# Autodesk Inventor assembly: Shoulder_r1
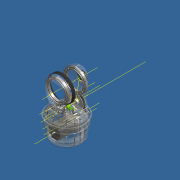
[picture p0: Inventor's stored thumbnail of the model, 180x180]
Saved by Autodesk Inventor 2016 (Build 200138000, 138)
## iProperties
Created: 2015-01-06
Part Number: Shoulder_r1
Document SubType Name: Assembly
Designer: 4ndreas
Mass: 7957.81 g
Surface Area: 6736.07 cm^2
Volume: 2402.06 cm^3
Density: 3.31292 g/cm^3
Parent: R1
Author: 4ndreas
## Documents named in this file (35)
- C:\Users\4ndreas\Documents\github\Mantis-Robot-Arm\MantisRobotArm\Workspace\_assemblys\Shoulder_r1.iam
- C:\Users\4ndreas\Documents\github\Mantis-Robot-Arm\MantisRobotArm\Workspace\_assemblys\Shoulder\Konstruktions-Assistent\Übertragung des Zahnriemens1.iam
- C:\Users\4ndreas\Documents\github\Mantis-Robot-Arm\MantisRobotArm\Libraries\Content Center Files\de-DE\DIN 125-1  A\DIN 125 - A 4,3.ipt
- C:\Users\4ndreas\Documents\github\Mantis-Robot-Arm\MantisRobotArm\Libraries\Content Center Files\de-DE\DIN BEARING(1)\DIN 625 SKF - SKF 624.ipt
- C:\Users\4ndreas\Documents\github\Mantis-Robot-Arm\MantisRobotArm\Libraries\Content Center Files\de-DE\DIN 934\DIN 934 - M4 x 0,7.ipt
- C:\Users\4ndreas\Documents\github\Mantis-Robot-Arm\MantisRobotArm\Workspace\_assemblys\Shoulder\Konstruktions-Assisten2\Übertragung des Zahnriemens1.iam
- C:\Users\4ndreas\Documents\github\Mantis-Robot-Arm\MantisRobotArm\Libraries\Content Center Files\de-DE\DIN BEARING(1)\DIN 625 SKF - SKF 61818.ipt
- C:\Users\4ndreas\Documents\github\Mantis-Robot-Arm\MantisRobotArm\Workspace\_misc parts\Shoulder_basis_N24.ipt
- C:\Users\4ndreas\Documents\github\Mantis-Robot-Arm\MantisRobotArm\Workspace\_assemblys\Shoulder\Konstruktions-Assistent\Welle1.iam
- C:\Users\4ndreas\Documents\github\Mantis-Robot-Arm\MantisRobotArm\Libraries\Content Center Files\de-DE\DIN BEARING(1)\DIN 625 SKF - SKF 608.ipt
- C:\Users\4ndreas\Documents\github\Mantis-Robot-Arm\MantisRobotArm\Libraries\Content Center Files\de-DE\DIN 125-1  A\DIN 125 - A 8,4.ipt
- C:\Users\4ndreas\Documents\github\Mantis-Robot-Arm\MantisRobotArm\Workspace\_printed parts\LagerKlemme.ipt
- C:\Users\4ndreas\Documents\github\Mantis-Robot-Arm\MantisRobotArm\Workspace\_metal parts\16221600.ipt
- C:\Users\4ndreas\Documents\github\Mantis-Robot-Arm\MantisRobotArm\Workspace\_metal parts\Synchrone RiemenscheibeT5_z48.ipt
- C:\Users\4ndreas\Documents\github\Mantis-Robot-Arm\MantisRobotArm\Workspace\_metal parts\Alu_Belt_tens.ipt
- C:\Users\4ndreas\Documents\github\Mantis-Robot-Arm\MantisRobotArm\Libraries\Content Center Files\de-DE\DIN 9021\DIN 9021 - 4,3.ipt
- C:\Users\4ndreas\Documents\github\Mantis-Robot-Arm\MantisRobotArm\Workspace\_standard Parts\DIN 912 - M4 x 0,7 x50.ipt
- C:\Users\4ndreas\Documents\github\Mantis-Robot-Arm\MantisRobotArm\Libraries\Content Center Files\de-DE\DIN 912\DIN 912 - M4 x 0,7 x 20 x 18,25.ipt
- C:\Users\4ndreas\Documents\github\Mantis-Robot-Arm\MantisRobotArm\Libraries\Content Center Files\de-DE\DIN 562\DIN 562 - M4 x 7.ipt
- C:\Users\4ndreas\Documents\github\Mantis-Robot-Arm\MantisRobotArm\Libraries\Content Center Files\de-DE\DIN 912\DIN 912 - M4 x 0,7 x 30 x 20.ipt
- C:\Users\4ndreas\Documents\github\Mantis-Robot-Arm\MantisRobotArm\Workspace\_standard Parts\DIN 912 - M4 x 0,7 x 60.ipt
- C:\Users\4ndreas\Documents\github\Mantis-Robot-Arm\MantisRobotArm\Libraries\Content Center Files\de-DE\DIN 7991(2)\DIN 7991 - M3x25.ipt
- C:\Users\4ndreas\Documents\github\Mantis-Robot-Arm\MantisRobotArm\Libraries\Content Center Files\de-DE\DIN 934\DIN 934 - M3 x 0,5.ipt
- C:\Users\4ndreas\Documents\github\Mantis-Robot-Arm\MantisRobotArm\Libraries\Content Center Files\de-DE\DIN 912\DIN 912 - M4 x 0,7 x 40 x 20.ipt
- C:\Users\4ndreas\Documents\github\Mantis-Robot-Arm\MantisRobotArm\Workspace\_standard Parts\Distanzhuelse_M4x20mm.ipt
- C:\Users\4ndreas\Documents\github\Mantis-Robot-Arm\MantisRobotArm\Libraries\Content Center Files\de-DE\DIN 913\DIN 913 - M4 x 4.ipt
- C:\Users\4ndreas\Documents\github\Mantis-Robot-Arm\MantisRobotArm\Libraries\Content Center Files\de-DE\BS EN ISO 13337\ISO 13337 - 3 x 20BS EN ISO.ipt
- C:\Users\4ndreas\Documents\github\Mantis-Robot-Arm\MantisRobotArm\Libraries\Content Center Files\de-DE\BS EN ISO 13337\ISO 13337 - 3 x 26BS EN ISO.ipt
- C:\Users\4ndreas\Documents\github\Mantis-Robot-Arm\MantisRobotArm\Libraries\Content Center Files\de-DE\DIN 711\DIN 711 - 511 20 - 100 x 135 x 25.ipt
- C:\Users\4ndreas\Documents\github\Mantis-Robot-Arm\MantisRobotArm\Workspace\_printed parts\CoverBase_r1.ipt
- C:\Users\4ndreas\Documents\github\Mantis-Robot-Arm\MantisRobotArm\Workspace\_standard Parts\bearing 6830 150x190x20 .ipt
- C:\Users\4ndreas\Documents\github\Mantis-Robot-Arm\MantisRobotArm\Workspace\_motors\Nema24_100.ipt
- C:\Users\4ndreas\Documents\github\Mantis-Robot-Arm\MantisRobotArm\Workspace\_encoder\encoderR1_mini.ipt
- C:\Users\4ndreas\Documents\github\Mantis-Robot-Arm\MantisRobotArm\Workspace\_encoder\encoder_neu.iam
- C:\Users\4ndreas\Documents\github\Mantis-Robot-Arm\MantisRobotArm\Workspace\_metal parts\Nema23_24Mount.ipt
## Components (139 placed, 32 different names)
1. Übertragung des Zahnriemens:1 [sub-assembly] — Passend:1, Passend:12, Passend:49, Passend:138, Fluchtend:18, Passend:147, Passend:173, Passend:195, Passend:228, Passend:229, Passend:410, Passend:411, Passend:422
2. DIN 912 - ersetzt durch DIN EN ISO 4762 M4 x 50:1 — Passend:69, Passend:82, Passend:99, Passend:179, Passend:198, Passend:203, Passend:209, Passend:210
3. DIN 625 SKF SKF 624:1 — Passend:178, Passend:192
4. DIN 625 SKF SKF 624:2 — Passend:177, Passend:186, Passend:188
5. DIN 625 SKF SKF 624:3 — Passend:80, Passend:82, Passend:181
6. DIN 625 SKF SKF 624:4 — Passend:80, Passend:180, Passend:212
7. DIN 125-1 A A 4,3:3 — Passend:193, Passend:219
8. DIN 125-1 A A 4,3:4 — Passend:183
9. DIN 125-1 A A 4,3:6 — Passend:189, Passend:194
10. DIN 934 - ersetzt durch DIN EN 24032/28673/28674 M4:1 — Passend:99, Passend:183
11. Übertragung des Zahnriemens:2 [sub-assembly] — Passend:130, Passend:182
12. Nema24_100:1 — Passend:130, Winkel:10, Passend:174, Passend:175, Passend:255, Passend:459, Passend:460, Passend:464, Passend:465, Passend:466, Passend:467, Passend:469, Passend:471
13. DIN 625 SKF SKF 61818:1 — Passend:138, Passend:142
14. DIN 625 SKF SKF 61818:2 — Passend:144, Fluchtend:17
15. Shoulder_basis_N24:1 — Passend:139, Fluchtend:14, Passend:140, Fluchtend:16, Passend:142, Passend:143, Passend:144, Fluchtend:17, Passend:164, Passend:169, Fluchtend:19, Passend:182, Passend:69, Passend:191, Fluchtend:20, Passend:204, Passend:205, Passend:206, Passend:208, Passend:213, Passend:221, Passend:224, Passend:225, Passend:226, Passend:227, Passend:230, Passend:300, Passend:301, Passend:302, Passend:303, Passend:304, Passend:305, Passend:306, Passend:307, Passend:308, Passend:309, Passend:310, Passend:311, Passend:328, Passend:329, Passend:330, Passend:331, Passend:332, Passend:333, Passend:334, Passend:335, Passend:336, Passend:337, Passend:338, Passend:339, Passend:340, Passend:341, Passend:342, Passend:344, Passend:345, Passend:346, Passend:353, Passend:354, Passend:355, Passend:356, Passend:357, Passend:358, Passend:359, Passend:367, Passend:369, Passend:370, Passend:371, Passend:374, Passend:375, Fluchtend:52, Fluchtend:53, Passend:423, Passend:424, Passend:425, Passend:426, Passend:448, Passend:449, Passend:450, Passend:451, Passend:456
16. CoverBase_r1:1 — Passend:143, Passend:164, Passend:230, Passend:239, Passend:240, Passend:241, Passend:242, Passend:247, Passend:248, Passend:249, Passend:250, Passend:255, Passend:257, Passend:258, Passend:261, Passend:262, Passend:263, Passend:264, Passend:377, Passend:384, Passend:391, Passend:393, Passend:413, Passend:414, Passend:415, Passend:416, Passend:418, Passend:419, Passend:420, Passend:421, Passend:427, Passend:430, Passend:457, Passend:458, Passend:463, Passend:472
17. Welle:1 [sub-assembly] — Fluchtend:18, Passend:147, Passend:153, Passend:154, Passend:155, Passend:165, Passend:166
18. DIN 625 SKF SKF 608:1 — Passend:153, Passend:167, Passend:169
19. DIN 625 SKF SKF 608:3 — Passend:154, Passend:170, Passend:171
20. DIN 625 SKF SKF 608:4 — Passend:155
21. Synchrone RiemenscheibeT5_z48:1 — Passend:165, Passend:172, Passend:407, Passend:408
22. DIN 125-1 A A 8,4:1 — Passend:166, Passend:167, Passend:172
23. DIN 125-1 A A 8,4:2 — Passend:170, Passend:171, Passend:173
24. LagerKlemme:1 — Fluchtend:19, Passend:226, Passend:227, Passend:324, Passend:325, Passend:326, Passend:327
25. 16221600:1 — Passend:174, Passend:175, Passend:409
26. DIN 625 SKF SKF 624:5 — Passend:177, Passend:178, Passend:190
27. DIN 625 SKF SKF 624:6 — Passend:179, Passend:180, Passend:181
28. Alu_Belt_tens:1 — Passend:186, Passend:191, Passend:196, Passend:197, Fluchtend:20, Passend:222
29. DIN 912 - ersetzt durch DIN EN ISO 4762 M4 x 20:1 — Passend:197, Passend:200, Passend:201
30. DIN 912 - ersetzt durch DIN EN ISO 4762 M4 x 20:2 — Passend:196, Passend:199, Passend:202
31. DIN 912 - ersetzt durch DIN EN ISO 4762 M4 x 40:9 — Passend:188, Passend:189, Passend:190, Passend:192, Passend:193, Passend:194, Passend:195, Passend:207, Passend:218
32. DIN 9021 4,3:1 — Passend:198, Passend:203, Passend:204
33. DIN 9021 4,3:2 — Passend:200, Passend:201, Passend:205
34. DIN 9021 4,3:3 — Passend:199, Passend:202, Passend:206
35. DIN 9021 4,3:4 — Passend:207, Passend:208, Passend:220
36. DIN 9021 4,3:5 — Passend:209, Passend:211, Passend:213
37. DIN 934 - ersetzt durch DIN EN 24032/28673/28674 M4:2 — Passend:210, Passend:211, Passend:212
38. DIN 125-1 A A 4,3:7 — Passend:215, Passend:217, Passend:220
39. DIN 125-1 A A 4,3:8 — Passend:214, Passend:215, Passend:216
40. DIN 125-1 A A 4,3:9 — Passend:214, Passend:216, Passend:217, Passend:218, Passend:219
41. DIN 912 - ersetzt durch DIN EN ISO 4762 M4 x 20:3 — Passend:221, Passend:222, Passend:223
42. DIN 934 - ersetzt durch DIN EN 24032/28673/28674 M4:3 — Passend:223, Passend:224, Passend:225
43. DIN 912 - ersetzt durch DIN EN ISO 4762 M4 x 20:4 — Passend:235, Passend:245, Passend:470, Passend:471
44. DIN 912 - ersetzt durch DIN EN ISO 4762 M4 x 20:5 — Passend:237, Passend:243, Passend:468, Passend:469
45. DIN 912 - ersetzt durch DIN EN ISO 4762 M4 x 20:6 — Passend:236, Passend:244
46. DIN 912 - ersetzt durch DIN EN ISO 4762 M4 x 20:7 — Passend:238, Passend:246
47. DIN 125-1 A A 4,3:10 — Passend:238, Passend:239, Passend:246
48. DIN 125-1 A A 4,3:11 — Passend:237, Passend:241, Passend:243
49. DIN 125-1 A A 4,3:12 — Passend:235, Passend:242, Passend:245
50. DIN 125-1 A A 4,3:13 — Passend:236, Passend:240, Passend:244
51. DIN 625 SKF SKF 624:7 — Passend:248, Passend:251, Passend:252
52. DIN 625 SKF SKF 624:8 — Passend:247, Passend:251, Passend:253, Passend:254
53. DIN 125-1 A A 4,3:14 — Passend:249, Passend:250, Passend:252
54. DIN 125-1 A A 4,3:15 — Passend:253, Passend:254
55. DIN 912 - ersetzt durch DIN EN ISO 4762 M4 x 50:9 — Passend:263, Passend:314, Fluchtend:51
56. DIN 912 - ersetzt durch DIN EN ISO 4762 M4 x 40:1 — Passend:262, Passend:313, Passend:384
57. DIN 912 - ersetzt durch DIN EN ISO 4762 M4 x 50:10 — Passend:261, Fluchtend:28, Passend:312
58. DIN 912 - ersetzt durch DIN EN ISO 4762 M4 x 30:5 — Passend:258, Passend:316, Passend:472
59. DIN 912 - ersetzt durch DIN EN ISO 4762 M4 x 50:13 — Passend:257, Fluchtend:28, Passend:317, Passend:377, Fluchtend:59
60. DIN 912 - ersetzt durch DIN EN ISO 4762 M4 x 50:17 — Passend:264, Passend:315, Fluchtend:51, Fluchtend:59
61. DIN 562 M4:1 — Passend:300, Passend:301, Passend:317
62. DIN 562 M4:2 — Passend:302, Passend:303, Passend:316
63. DIN 562 M4:3 — Passend:304, Passend:305, Passend:315
64. DIN 562 M4:4 — Passend:307, Passend:310, Passend:313
65. DIN 562 M4:5 — Passend:306, Passend:311, Passend:312
66. DIN 562 M4:6 — Passend:308, Passend:309, Passend:314
67. DIN 912 - ersetzt durch DIN EN ISO 4762 M4 x 30:1 — Passend:318, Passend:321, Passend:322, Passend:324
68. DIN 912 - ersetzt durch DIN EN ISO 4762 M4 x 30:2 — Passend:319, Passend:320, Passend:323, Passend:326
69. DIN 934 - ersetzt durch DIN EN 24032/28673/28674 M4:12 — Passend:319, Fluchtend:43, Passend:329
70. DIN 934 - ersetzt durch DIN EN 24032/28673/28674 M4:13 — Passend:318, Fluchtend:43, Passend:328, Passend:330
71. DIN 125-1 A A 4,3:16 — Passend:321, Passend:322, Passend:325
72. DIN 125-1 A A 4,3:17 — Passend:320, Passend:323, Passend:327
73. Distanzhuelse_M4x20mm:9 — Passend:333, Passend:339, Passend:342, Passend:347
74. Distanzhuelse_M4x20mm:10 — Passend:334, Passend:340, Passend:341, Passend:351
75. Distanzhuelse_M4x20mm:11 — Passend:331, Passend:335, Passend:338, Passend:349
76. Distanzhuelse_M4x20mm:12 — Passend:332, Passend:336, Passend:337
77. DIN 912 - ersetzt durch DIN EN ISO 4762 M4 x 50:2 — Passend:344, Passend:346
78. DIN 912 - ersetzt durch DIN EN ISO 4762 M4 x 50:3 — Passend:347, Passend:348, Passend:359
79. DIN 912 - ersetzt durch DIN EN ISO 4762 M4 x 50:4 — Passend:348, Passend:353
80. DIN 912 - ersetzt durch DIN EN ISO 4762 M4 x 50:5 — Passend:345, Passend:356
81. DIN 912 - ersetzt durch DIN EN ISO 4762 M4 x 60:16 — Passend:350, Passend:355
82. DIN 912 - ersetzt durch DIN EN ISO 4762 M4 x 60:17 — Passend:349, Passend:350, Passend:357
83. DIN 912 - ersetzt durch DIN EN ISO 4762 M4 x 60:18 — Passend:352, Passend:354
84. DIN 912 - ersetzt durch DIN EN ISO 4762 M4 x 60:19 — Passend:351, Passend:352, Passend:358
85. DIN 912 - ersetzt durch DIN EN ISO 4762 M4 x 40:8 — Passend:386, Passend:388, Passend:389, Passend:390, Passend:391
86. DIN 125-1 A A 4,3:18 — Passend:386, Passend:390, Passend:463
87. DIN 9021 4,3:6 — Passend:387, Passend:388, Passend:393
88. DIN 934 - ersetzt durch DIN EN 24032/28673/28674 M4:14 — Passend:387, Passend:389
89. DIN 913 M4 x 4:1 — Passend:409
90. DIN 913 M4 x 4:2 — Passend:408
91. BS EN ISO 13337 3 x 20:1 — Passend:410
92. BS EN ISO 13337 3 x 26:1 — Passend:407
93. DIN 913 M4 x 4:3 — Passend:411
94. DIN 711 511 20 - 100 x 135 x 25:1 — Passend:413, Passend:414
95. DIN 625 SKF SKF 61818:3 — Passend:415, Passend:416
96. encoderR1_mini:1 — Passend:418, Passend:420, Passend:421
97. encoder_neu:1 [sub-assembly] — Passend:422, Passend:423, Passend:424
98. DIN 912 - ersetzt durch DIN EN ISO 4762 M4 x 60:1 — Passend:425, Passend:426, Fluchtend:62, Fluchtend:66
99. DIN 912 - ersetzt durch DIN EN ISO 4762 M4 x 40:2 — Passend:427, Passend:431
100. DIN 9021 4,3:11 — Passend:430, Fluchtend:61, Fluchtend:73, Fluchtend:74, Fluchtend:75
101. Distanzhuelse_M4x20mm:13 — Passend:431, Fluchtend:60, Fluchtend:67, Fluchtend:68
102. DIN 912 - ersetzt durch DIN EN ISO 4762 M4 x 60:20 — Passend:435, Fluchtend:62, Passend:448
103. DIN 912 - ersetzt durch DIN EN ISO 4762 M4 x 40:3
104. DIN 9021 4,3:12 — Fluchtend:61, Fluchtend:74
105. Distanzhuelse_M4x20mm:14 — Passend:435, Fluchtend:60
106. DIN 912 - ersetzt durch DIN EN ISO 4762 M4 x 60:21 — Passend:451, Fluchtend:64, Fluchtend:65
107. DIN 912 - ersetzt durch DIN EN ISO 4762 M4 x 40:4
108. DIN 9021 4,3:13 — Fluchtend:71
109. Distanzhuelse_M4x20mm:15 — Fluchtend:70
110. DIN 912 - ersetzt durch DIN EN ISO 4762 M4 x 60:22 — Passend:450, Fluchtend:63
111. DIN 912 - ersetzt durch DIN EN ISO 4762 M4 x 40:5
112. DIN 9021 4,3:14 — Fluchtend:72, Fluchtend:73
113. Distanzhuelse_M4x20mm:16 — Fluchtend:69
114. DIN 912 - ersetzt durch DIN EN ISO 4762 M4 x 60:23 — Passend:449, Fluchtend:65, Fluchtend:66
115. DIN 912 - ersetzt durch DIN EN ISO 4762 M4 x 40:6
116. DIN 9021 4,3:15 — Fluchtend:75
117. Distanzhuelse_M4x20mm:17 — Fluchtend:67
118. DIN 912 - ersetzt durch DIN EN ISO 4762 M4 x 60:24 — Passend:456, Fluchtend:63, Fluchtend:64
119. DIN 912 - ersetzt durch DIN EN ISO 4762 M4 x 40:7
120. DIN 9021 4,3:16 — Fluchtend:71, Fluchtend:72
121. Distanzhuelse_M4x20mm:18 — Fluchtend:68, Fluchtend:69, Fluchtend:70
122. DIN 912 - ersetzt durch DIN EN ISO 4762 M4 x 30:3 — Passend:458, Passend:460, Passend:461
123. DIN 912 - ersetzt durch DIN EN ISO 4762 M4 x 30:4 — Passend:457, Passend:459, Passend:462
124. DIN 934 - ersetzt durch DIN EN 24032/28673/28674 M4:19 — Passend:461, Fluchtend:76, Fluchtend:77
125. DIN 934 - ersetzt durch DIN EN 24032/28673/28674 M4:20 — Passend:462, Fluchtend:76, Fluchtend:77
126. Nema23_24Mount:1 — Passend:464, Passend:465, Passend:466
127. Nema23_24Mount:2 — Passend:467, Passend:468, Passend:470
128. DIN 934 - ersetzt durch DIN EN 24032/28673/28674 M3:1 — Passend:368, Passend:369, Passend:370
129. DIN 7991 M3x25:1 — Passend:367, Fluchtend:52, Passend:368
130. DIN 934 - ersetzt durch DIN EN 24032/28673/28674 M3:2
131. DIN 7991 M3x25:2
132. DIN 934 - ersetzt durch DIN EN 24032/28673/28674 M3:3
133. DIN 7991 M3x25:3
134. DIN 7991 M3x25:8 — Passend:371, Passend:373, Fluchtend:53
135. DIN 934 - ersetzt durch DIN EN 24032/28673/28674 M3:8 — Passend:373, Passend:374, Passend:375
136. DIN 7991 M3x25:9
137. DIN 934 - ersetzt durch DIN EN 24032/28673/28674 M3:9
138. DIN 7991 M3x25:10
139. DIN 934 - ersetzt durch DIN EN 24032/28673/28674 M3:10
## Component patterns: (3 elements, first: DIN 934 - ersetzt durch DIN EN 24032/28673/28674 M3:1 + DIN 7991 M3x25:1), (3 elements, first: DIN 7991 M3x25:8 + DIN 934 - ersetzt durch DIN EN 24032/28673/28674 M3:8)
## Relationships (287: Mate 254, Flush 32, Angle 1)
- Passend:1 [Mate]: Übertragung des Zahnriemens:1
- Passend:4 [Mate]
- Passend:12 [Mate]: Übertragung des Zahnriemens:1
- Passend:49 [Mate]: Übertragung des Zahnriemens:1
- Passend:62 [Mate]
- Passend:63 [Mate]
- Passend:69 [Mate]: DIN 912 - ersetzt durch DIN EN ISO 4762 M4 x 50:1 ↔ Shoulder_basis_N24:1
- Passend:80 [Mate]: DIN 625 SKF SKF 624:3 ↔ DIN 625 SKF SKF 624:4
- Passend:82 [Mate]: DIN 912 - ersetzt durch DIN EN ISO 4762 M4 x 50:1 ↔ DIN 625 SKF SKF 624:3
- [Mate]: DIN 912 - ersetzt durch DIN EN ISO 4762 M4 x 50:1 ↔ DIN 125-1 A A 4,3:4
- [Mate]: DIN 625 SKF SKF 624:3 ↔ DIN 125-1 A A 4,3:4
- [Mate]: DIN 625 SKF SKF 624:2 ↔ DIN 125-1 A A 4,3:6
- [Mate]: DIN 625 SKF SKF 624:1 ↔ DIN 125-1 A A 4,3:3
- Passend:99 [Mate]: DIN 912 - ersetzt durch DIN EN ISO 4762 M4 x 50:1 ↔ DIN 934 - ersetzt durch DIN EN 24032/28673/28674 M4:1
- Fluchtend:12 [Flush] (43 mm)
- Fluchtend:13 [Flush] (20 mm)
- Passend:130 [Mate]: Übertragung des Zahnriemens:2 ↔ Nema24_100:1
- Winkel:10 [Angle] (0 deg): Nema24_100:1
- Passend:138 [Mate]: Übertragung des Zahnriemens:1 ↔ DIN 625 SKF SKF 61818:1
- Passend:139 [Mate]: Shoulder_basis_N24:1
- Fluchtend:14 [Flush]: Shoulder_basis_N24:1
- Passend:140 [Mate]: Shoulder_basis_N24:1
- Fluchtend:16 [Flush]: Shoulder_basis_N24:1
- Passend:142 [Mate]: DIN 625 SKF SKF 61818:1 ↔ Shoulder_basis_N24:1
- Passend:143 [Mate]: Shoulder_basis_N24:1 ↔ CoverBase_r1:1
- Passend:144 [Mate]: DIN 625 SKF SKF 61818:2 ↔ Shoulder_basis_N24:1
- Fluchtend:17 [Flush]: DIN 625 SKF SKF 61818:2 ↔ Shoulder_basis_N24:1
- Fluchtend:18 [Flush] (-10 mm): Übertragung des Zahnriemens:1 ↔ Welle:1
- Passend:147 [Mate]: Übertragung des Zahnriemens:1 ↔ Welle:1
- Passend:153 [Mate]: Welle:1 ↔ DIN 625 SKF SKF 608:1
- Passend:154 [Mate]: Welle:1 ↔ DIN 625 SKF SKF 608:3
- Passend:155 [Mate]: Welle:1 ↔ DIN 625 SKF SKF 608:4
- Passend:164 [Mate]: Shoulder_basis_N24:1 ↔ CoverBase_r1:1
- Passend:165 [Mate]: Welle:1 ↔ Synchrone RiemenscheibeT5_z48:1
- Passend:166 [Mate]: Welle:1 ↔ DIN 125-1 A A 8,4:1
- Passend:167 [Mate]: DIN 625 SKF SKF 608:1 ↔ DIN 125-1 A A 8,4:1
- Passend:169 [Mate]: Shoulder_basis_N24:1 ↔ DIN 625 SKF SKF 608:1
- Passend:170 [Mate]: DIN 625 SKF SKF 608:3 ↔ DIN 125-1 A A 8,4:2
- Passend:171 [Mate]: DIN 625 SKF SKF 608:3 ↔ DIN 125-1 A A 8,4:2
- Passend:172 [Mate]: Synchrone RiemenscheibeT5_z48:1 ↔ DIN 125-1 A A 8,4:1
- Passend:173 [Mate] (0.5 mm): Übertragung des Zahnriemens:1 ↔ DIN 125-1 A A 8,4:2
- Fluchtend:19 [Flush]: Shoulder_basis_N24:1 ↔ LagerKlemme:1
- Passend:174 [Mate]: Nema24_100:1 ↔ 16221600:1
- Passend:175 [Mate] (0.5 mm): Nema24_100:1 ↔ 16221600:1
- Passend:177 [Mate]: DIN 625 SKF SKF 624:2 ↔ DIN 625 SKF SKF 624:5
- Passend:178 [Mate]: DIN 625 SKF SKF 624:1 ↔ DIN 625 SKF SKF 624:5
- Passend:179 [Mate]: DIN 912 - ersetzt durch DIN EN ISO 4762 M4 x 50:1 ↔ DIN 625 SKF SKF 624:6
- Passend:180 [Mate]: DIN 625 SKF SKF 624:4 ↔ DIN 625 SKF SKF 624:6
- Passend:181 [Mate]: DIN 625 SKF SKF 624:3 ↔ DIN 625 SKF SKF 624:6
- Passend:182 [Mate]: Übertragung des Zahnriemens:2 ↔ Shoulder_basis_N24:1
- Passend:183 [Mate]: DIN 125-1 A A 4,3:4 ↔ DIN 934 - ersetzt durch DIN EN 24032/28673/28674 M4:1
- Passend:186 [Mate]: DIN 625 SKF SKF 624:2 ↔ Alu_Belt_tens:1
- Passend:188 [Mate]: DIN 625 SKF SKF 624:2 ↔ DIN 912 - ersetzt durch DIN EN ISO 4762 M4 x 40:9
- Passend:189 [Mate]: DIN 125-1 A A 4,3:6 ↔ DIN 912 - ersetzt durch DIN EN ISO 4762 M4 x 40:9
- Passend:190 [Mate]: DIN 625 SKF SKF 624:5 ↔ DIN 912 - ersetzt durch DIN EN ISO 4762 M4 x 40:9
- Passend:191 [Mate]: Shoulder_basis_N24:1 ↔ Alu_Belt_tens:1
- Passend:192 [Mate]: DIN 625 SKF SKF 624:1 ↔ DIN 912 - ersetzt durch DIN EN ISO 4762 M4 x 40:9
- Passend:193 [Mate]: DIN 125-1 A A 4,3:3 ↔ DIN 912 - ersetzt durch DIN EN ISO 4762 M4 x 40:9
- Passend:194 [Mate]: DIN 125-1 A A 4,3:6 ↔ DIN 912 - ersetzt durch DIN EN ISO 4762 M4 x 40:9
- Passend:195 [Mate]: Übertragung des Zahnriemens:1 ↔ DIN 912 - ersetzt durch DIN EN ISO 4762 M4 x 40:9
- Passend:196 [Mate]: Alu_Belt_tens:1 ↔ DIN 912 - ersetzt durch DIN EN ISO 4762 M4 x 20:2
- Passend:197 [Mate]: Alu_Belt_tens:1 ↔ DIN 912 - ersetzt durch DIN EN ISO 4762 M4 x 20:1
- Fluchtend:20 [Flush]: Shoulder_basis_N24:1 ↔ Alu_Belt_tens:1
- Passend:198 [Mate]: DIN 912 - ersetzt durch DIN EN ISO 4762 M4 x 50:1 ↔ DIN 9021 4,3:1
- Passend:199 [Mate]: DIN 912 - ersetzt durch DIN EN ISO 4762 M4 x 20:2 ↔ DIN 9021 4,3:3
- Passend:200 [Mate]: DIN 912 - ersetzt durch DIN EN ISO 4762 M4 x 20:1 ↔ DIN 9021 4,3:2
- Passend:201 [Mate]: DIN 912 - ersetzt durch DIN EN ISO 4762 M4 x 20:1 ↔ DIN 9021 4,3:2
- Passend:202 [Mate]: DIN 912 - ersetzt durch DIN EN ISO 4762 M4 x 20:2 ↔ DIN 9021 4,3:3
- Passend:203 [Mate]: DIN 912 - ersetzt durch DIN EN ISO 4762 M4 x 50:1 ↔ DIN 9021 4,3:1
- Passend:204 [Mate]: Shoulder_basis_N24:1 ↔ DIN 9021 4,3:1
- Passend:205 [Mate]: Shoulder_basis_N24:1 ↔ DIN 9021 4,3:2
- Passend:206 [Mate]: Shoulder_basis_N24:1 ↔ DIN 9021 4,3:3
- Passend:207 [Mate]: DIN 912 - ersetzt durch DIN EN ISO 4762 M4 x 40:9 ↔ DIN 9021 4,3:4
- Passend:208 [Mate]: Shoulder_basis_N24:1 ↔ DIN 9021 4,3:4
- Passend:209 [Mate]: DIN 912 - ersetzt durch DIN EN ISO 4762 M4 x 50:1 ↔ DIN 9021 4,3:5
- Passend:210 [Mate]: DIN 912 - ersetzt durch DIN EN ISO 4762 M4 x 50:1 ↔ DIN 934 - ersetzt durch DIN EN 24032/28673/28674 M4:2
- Passend:211 [Mate]: DIN 9021 4,3:5 ↔ DIN 934 - ersetzt durch DIN EN 24032/28673/28674 M4:2
- Passend:212 [Mate]: DIN 625 SKF SKF 624:4 ↔ DIN 934 - ersetzt durch DIN EN 24032/28673/28674 M4:2
- Passend:213 [Mate]: Shoulder_basis_N24:1 ↔ DIN 9021 4,3:5
- Passend:214 [Mate]: DIN 125-1 A A 4,3:8 ↔ DIN 125-1 A A 4,3:9
- Passend:215 [Mate]: DIN 125-1 A A 4,3:7 ↔ DIN 125-1 A A 4,3:8
- Passend:216 [Mate]: DIN 125-1 A A 4,3:8 ↔ DIN 125-1 A A 4,3:9
- Passend:217 [Mate]: DIN 125-1 A A 4,3:7 ↔ DIN 125-1 A A 4,3:9
- Passend:218 [Mate]: DIN 912 - ersetzt durch DIN EN ISO 4762 M4 x 40:9 ↔ DIN 125-1 A A 4,3:9
- Passend:219 [Mate]: DIN 125-1 A A 4,3:3 ↔ DIN 125-1 A A 4,3:9
- Passend:220 [Mate]: DIN 9021 4,3:4 ↔ DIN 125-1 A A 4,3:7
- Passend:221 [Mate]: Shoulder_basis_N24:1 ↔ DIN 912 - ersetzt durch DIN EN ISO 4762 M4 x 20:3
- Passend:222 [Mate]: Alu_Belt_tens:1 ↔ DIN 912 - ersetzt durch DIN EN ISO 4762 M4 x 20:3
- Passend:223 [Mate]: DIN 912 - ersetzt durch DIN EN ISO 4762 M4 x 20:3 ↔ DIN 934 - ersetzt durch DIN EN 24032/28673/28674 M4:3
- Passend:224 [Mate]: Shoulder_basis_N24:1 ↔ DIN 934 - ersetzt durch DIN EN 24032/28673/28674 M4:3
- Passend:225 [Mate]: Shoulder_basis_N24:1 ↔ DIN 934 - ersetzt durch DIN EN 24032/28673/28674 M4:3
- Passend:226 [Mate]: Shoulder_basis_N24:1 ↔ LagerKlemme:1
- Passend:227 [Mate]: Shoulder_basis_N24:1 ↔ LagerKlemme:1
- Passend:228 [Mate]: Übertragung des Zahnriemens:1
- Passend:229 [Mate]: Übertragung des Zahnriemens:1
- Passend:230 [Mate]: Shoulder_basis_N24:1 ↔ CoverBase_r1:1
- Passend:235 [Mate]: DIN 912 - ersetzt durch DIN EN ISO 4762 M4 x 20:4 ↔ DIN 125-1 A A 4,3:12
- Passend:236 [Mate]: DIN 912 - ersetzt durch DIN EN ISO 4762 M4 x 20:6 ↔ DIN 125-1 A A 4,3:13
- Passend:237 [Mate]: DIN 912 - ersetzt durch DIN EN ISO 4762 M4 x 20:5 ↔ DIN 125-1 A A 4,3:11
- Passend:238 [Mate]: DIN 912 - ersetzt durch DIN EN ISO 4762 M4 x 20:7 ↔ DIN 125-1 A A 4,3:10
- Passend:239 [Mate]: CoverBase_r1:1 ↔ DIN 125-1 A A 4,3:10
- Passend:240 [Mate]: CoverBase_r1:1 ↔ DIN 125-1 A A 4,3:13
- Passend:241 [Mate]: CoverBase_r1:1 ↔ DIN 125-1 A A 4,3:11
- Passend:242 [Mate]: CoverBase_r1:1 ↔ DIN 125-1 A A 4,3:12
- Passend:243 [Mate]: DIN 912 - ersetzt durch DIN EN ISO 4762 M4 x 20:5 ↔ DIN 125-1 A A 4,3:11
- Passend:244 [Mate]: DIN 912 - ersetzt durch DIN EN ISO 4762 M4 x 20:6 ↔ DIN 125-1 A A 4,3:13
- Passend:245 [Mate]: DIN 912 - ersetzt durch DIN EN ISO 4762 M4 x 20:4 ↔ DIN 125-1 A A 4,3:12
- Passend:246 [Mate]: DIN 912 - ersetzt durch DIN EN ISO 4762 M4 x 20:7 ↔ DIN 125-1 A A 4,3:10
- Passend:247 [Mate]: CoverBase_r1:1 ↔ DIN 625 SKF SKF 624:8
- Passend:248 [Mate]: CoverBase_r1:1 ↔ DIN 625 SKF SKF 624:7
- Passend:249 [Mate]: CoverBase_r1:1 ↔ DIN 125-1 A A 4,3:14
- Passend:250 [Mate]: CoverBase_r1:1 ↔ DIN 125-1 A A 4,3:14
- Passend:251 [Mate]: DIN 625 SKF SKF 624:7 ↔ DIN 625 SKF SKF 624:8
- Passend:252 [Mate]: DIN 625 SKF SKF 624:7 ↔ DIN 125-1 A A 4,3:14
- Passend:253 [Mate]: DIN 625 SKF SKF 624:8 ↔ DIN 125-1 A A 4,3:15
- Passend:254 [Mate]: DIN 625 SKF SKF 624:8 ↔ DIN 125-1 A A 4,3:15
- Passend:255 [Mate]: Nema24_100:1 ↔ CoverBase_r1:1
- Passend:257 [Mate]: CoverBase_r1:1 ↔ DIN 912 - ersetzt durch DIN EN ISO 4762 M4 x 50:13
- Passend:258 [Mate]: CoverBase_r1:1 ↔ DIN 912 - ersetzt durch DIN EN ISO 4762 M4 x 30:5
- Passend:261 [Mate]: CoverBase_r1:1 ↔ DIN 912 - ersetzt durch DIN EN ISO 4762 M4 x 50:10
- Passend:262 [Mate]: CoverBase_r1:1 ↔ DIN 912 - ersetzt durch DIN EN ISO 4762 M4 x 40:1
- Passend:263 [Mate]: CoverBase_r1:1 ↔ DIN 912 - ersetzt durch DIN EN ISO 4762 M4 x 50:9
- Passend:264 [Mate]: CoverBase_r1:1 ↔ DIN 912 - ersetzt durch DIN EN ISO 4762 M4 x 50:17
- Fluchtend:28 [Flush]: DIN 912 - ersetzt durch DIN EN ISO 4762 M4 x 50:10 ↔ DIN 912 - ersetzt durch DIN EN ISO 4762 M4 x 50:13
- Passend:300 [Mate]: Shoulder_basis_N24:1 ↔ DIN 562 M4:1
- Passend:301 [Mate]: Shoulder_basis_N24:1 ↔ DIN 562 M4:1
- Passend:302 [Mate]: Shoulder_basis_N24:1 ↔ DIN 562 M4:2
- Passend:303 [Mate]: Shoulder_basis_N24:1 ↔ DIN 562 M4:2
- Passend:304 [Mate]: Shoulder_basis_N24:1 ↔ DIN 562 M4:3
- Passend:305 [Mate]: Shoulder_basis_N24:1 ↔ DIN 562 M4:3
- Passend:306 [Mate]: Shoulder_basis_N24:1 ↔ DIN 562 M4:5
- Passend:307 [Mate]: Shoulder_basis_N24:1 ↔ DIN 562 M4:4
- Passend:308 [Mate]: Shoulder_basis_N24:1 ↔ DIN 562 M4:6
- Passend:309 [Mate]: Shoulder_basis_N24:1 ↔ DIN 562 M4:6
- Passend:310 [Mate]: Shoulder_basis_N24:1 ↔ DIN 562 M4:4
- Passend:311 [Mate]: Shoulder_basis_N24:1 ↔ DIN 562 M4:5
- Passend:312 [Mate]: DIN 912 - ersetzt durch DIN EN ISO 4762 M4 x 50:10 ↔ DIN 562 M4:5
- Passend:313 [Mate]: DIN 912 - ersetzt durch DIN EN ISO 4762 M4 x 40:1 ↔ DIN 562 M4:4
- Passend:314 [Mate]: DIN 912 - ersetzt durch DIN EN ISO 4762 M4 x 50:9 ↔ DIN 562 M4:6
- Passend:315 [Mate]: DIN 912 - ersetzt durch DIN EN ISO 4762 M4 x 50:17 ↔ DIN 562 M4:3
- Passend:316 [Mate]: DIN 912 - ersetzt durch DIN EN ISO 4762 M4 x 30:5 ↔ DIN 562 M4:2
- Passend:317 [Mate]: DIN 912 - ersetzt durch DIN EN ISO 4762 M4 x 50:13 ↔ DIN 562 M4:1
- Passend:318 [Mate]: DIN 912 - ersetzt durch DIN EN ISO 4762 M4 x 30:1 ↔ DIN 934 - ersetzt durch DIN EN 24032/28673/28674 M4:13
- Passend:319 [Mate]: DIN 912 - ersetzt durch DIN EN ISO 4762 M4 x 30:2 ↔ DIN 934 - ersetzt durch DIN EN 24032/28673/28674 M4:12
- Passend:320 [Mate]: DIN 912 - ersetzt durch DIN EN ISO 4762 M4 x 30:2 ↔ DIN 125-1 A A 4,3:17
- Passend:321 [Mate]: DIN 912 - ersetzt durch DIN EN ISO 4762 M4 x 30:1 ↔ DIN 125-1 A A 4,3:16
- Passend:322 [Mate]: DIN 912 - ersetzt durch DIN EN ISO 4762 M4 x 30:1 ↔ DIN 125-1 A A 4,3:16
- Passend:323 [Mate]: DIN 912 - ersetzt durch DIN EN ISO 4762 M4 x 30:2 ↔ DIN 125-1 A A 4,3:17
- Passend:324 [Mate]: LagerKlemme:1 ↔ DIN 912 - ersetzt durch DIN EN ISO 4762 M4 x 30:1
- Passend:325 [Mate]: LagerKlemme:1 ↔ DIN 125-1 A A 4,3:16
- Passend:326 [Mate]: LagerKlemme:1 ↔ DIN 912 - ersetzt durch DIN EN ISO 4762 M4 x 30:2
- Passend:327 [Mate]: LagerKlemme:1 ↔ DIN 125-1 A A 4,3:17
- Fluchtend:43 [Flush]: DIN 934 - ersetzt durch DIN EN 24032/28673/28674 M4:12 ↔ DIN 934 - ersetzt durch DIN EN 24032/28673/28674 M4:13
- Passend:328 [Mate]: Shoulder_basis_N24:1 ↔ DIN 934 - ersetzt durch DIN EN 24032/28673/28674 M4:13
- Passend:329 [Mate]: Shoulder_basis_N24:1 ↔ DIN 934 - ersetzt durch DIN EN 24032/28673/28674 M4:12
- Passend:330 [Mate]: Shoulder_basis_N24:1 ↔ DIN 934 - ersetzt durch DIN EN 24032/28673/28674 M4:13
- Passend:331 [Mate]: Shoulder_basis_N24:1 ↔ Distanzhuelse_M4x20mm:11
- Passend:332 [Mate]: Shoulder_basis_N24:1 ↔ Distanzhuelse_M4x20mm:12
- Passend:333 [Mate]: Shoulder_basis_N24:1 ↔ Distanzhuelse_M4x20mm:9
- Passend:334 [Mate]: Shoulder_basis_N24:1 ↔ Distanzhuelse_M4x20mm:10
- Passend:335 [Mate]: Shoulder_basis_N24:1 ↔ Distanzhuelse_M4x20mm:11
- Passend:336 [Mate]: Shoulder_basis_N24:1 ↔ Distanzhuelse_M4x20mm:12
- Passend:337 [Mate]: Shoulder_basis_N24:1 ↔ Distanzhuelse_M4x20mm:12
- Passend:338 [Mate]: Shoulder_basis_N24:1 ↔ Distanzhuelse_M4x20mm:11
- Passend:339 [Mate]: Shoulder_basis_N24:1 ↔ Distanzhuelse_M4x20mm:9
- Passend:340 [Mate]: Shoulder_basis_N24:1 ↔ Distanzhuelse_M4x20mm:10
- Passend:341 [Mate]: Shoulder_basis_N24:1 ↔ Distanzhuelse_M4x20mm:10
- Passend:342 [Mate]: Shoulder_basis_N24:1 ↔ Distanzhuelse_M4x20mm:9
- Passend:344 [Mate]: Shoulder_basis_N24:1 ↔ DIN 912 - ersetzt durch DIN EN ISO 4762 M4 x 50:2
- Passend:345 [Mate]: Shoulder_basis_N24:1 ↔ DIN 912 - ersetzt durch DIN EN ISO 4762 M4 x 50:5
- Passend:346 [Mate]: Shoulder_basis_N24:1 ↔ DIN 912 - ersetzt durch DIN EN ISO 4762 M4 x 50:2
- Passend:347 [Mate]: Distanzhuelse_M4x20mm:9 ↔ DIN 912 - ersetzt durch DIN EN ISO 4762 M4 x 50:3
- Passend:348 [Mate]: DIN 912 - ersetzt durch DIN EN ISO 4762 M4 x 50:3 ↔ DIN 912 - ersetzt durch DIN EN ISO 4762 M4 x 50:4
- Passend:349 [Mate]: Distanzhuelse_M4x20mm:11 ↔ DIN 912 - ersetzt durch DIN EN ISO 4762 M4 x 60:17
- Passend:350 [Mate]: DIN 912 - ersetzt durch DIN EN ISO 4762 M4 x 60:16 ↔ DIN 912 - ersetzt durch DIN EN ISO 4762 M4 x 60:17
- Passend:351 [Mate]: Distanzhuelse_M4x20mm:10 ↔ DIN 912 - ersetzt durch DIN EN ISO 4762 M4 x 60:19
- Passend:352 [Mate]: DIN 912 - ersetzt durch DIN EN ISO 4762 M4 x 60:18 ↔ DIN 912 - ersetzt durch DIN EN ISO 4762 M4 x 60:19
- Passend:353 [Mate]: Shoulder_basis_N24:1 ↔ DIN 912 - ersetzt durch DIN EN ISO 4762 M4 x 50:4
- Passend:354 [Mate]: Shoulder_basis_N24:1 ↔ DIN 912 - ersetzt durch DIN EN ISO 4762 M4 x 60:18
- Passend:355 [Mate]: Shoulder_basis_N24:1 ↔ DIN 912 - ersetzt durch DIN EN ISO 4762 M4 x 60:16
- Passend:356 [Mate]: Shoulder_basis_N24:1 ↔ DIN 912 - ersetzt durch DIN EN ISO 4762 M4 x 50:5
- Passend:357 [Mate]: Shoulder_basis_N24:1 ↔ DIN 912 - ersetzt durch DIN EN ISO 4762 M4 x 60:17
- Passend:358 [Mate]: Shoulder_basis_N24:1 ↔ DIN 912 - ersetzt durch DIN EN ISO 4762 M4 x 60:19
- Passend:359 [Mate]: Shoulder_basis_N24:1 ↔ DIN 912 - ersetzt durch DIN EN ISO 4762 M4 x 50:3
- Passend:367 [Mate]: Shoulder_basis_N24:1 ↔ DIN 7991 M3x25:1
- Fluchtend:52 [Flush]: Shoulder_basis_N24:1 ↔ DIN 7991 M3x25:1
- Passend:368 [Mate]: DIN 934 - ersetzt durch DIN EN 24032/28673/28674 M3:1 ↔ DIN 7991 M3x25:1
- Passend:369 [Mate]: Shoulder_basis_N24:1 ↔ DIN 934 - ersetzt durch DIN EN 24032/28673/28674 M3:1
- Passend:370 [Mate]: Shoulder_basis_N24:1 ↔ DIN 934 - ersetzt durch DIN EN 24032/28673/28674 M3:1
- Passend:371 [Mate]: Shoulder_basis_N24:1 ↔ DIN 7991 M3x25:8
- Passend:373 [Mate]: DIN 7991 M3x25:8 ↔ DIN 934 - ersetzt durch DIN EN 24032/28673/28674 M3:8
- Passend:374 [Mate]: Shoulder_basis_N24:1 ↔ DIN 934 - ersetzt durch DIN EN 24032/28673/28674 M3:8
- Passend:375 [Mate]: Shoulder_basis_N24:1 ↔ DIN 934 - ersetzt durch DIN EN 24032/28673/28674 M3:8
- Fluchtend:53 [Flush]: Shoulder_basis_N24:1 ↔ DIN 7991 M3x25:8
- Fluchtend:51 [Flush]: DIN 912 - ersetzt durch DIN EN ISO 4762 M4 x 50:9 ↔ DIN 912 - ersetzt durch DIN EN ISO 4762 M4 x 50:17
- Passend:377 [Mate]: CoverBase_r1:1 ↔ DIN 912 - ersetzt durch DIN EN ISO 4762 M4 x 50:13
- Passend:384 [Mate]: CoverBase_r1:1 ↔ DIN 912 - ersetzt durch DIN EN ISO 4762 M4 x 40:1
- Passend:386 [Mate]: DIN 912 - ersetzt durch DIN EN ISO 4762 M4 x 40:8 ↔ DIN 125-1 A A 4,3:18
- Passend:387 [Mate]: DIN 9021 4,3:6 ↔ DIN 934 - ersetzt durch DIN EN 24032/28673/28674 M4:14
- Passend:388 [Mate]: DIN 912 - ersetzt durch DIN EN ISO 4762 M4 x 40:8 ↔ DIN 9021 4,3:6
- Passend:389 [Mate]: DIN 912 - ersetzt durch DIN EN ISO 4762 M4 x 40:8 ↔ DIN 934 - ersetzt durch DIN EN 24032/28673/28674 M4:14
- Passend:390 [Mate]: DIN 912 - ersetzt durch DIN EN ISO 4762 M4 x 40:8 ↔ DIN 125-1 A A 4,3:18
- Passend:391 [Mate]: CoverBase_r1:1 ↔ DIN 912 - ersetzt durch DIN EN ISO 4762 M4 x 40:8
- Passend:393 [Mate]: CoverBase_r1:1 ↔ DIN 9021 4,3:6
- Passend:407 [Mate]: Synchrone RiemenscheibeT5_z48:1 ↔ BS EN ISO 13337 3 x 26:1
- Passend:408 [Mate]: Synchrone RiemenscheibeT5_z48:1 ↔ DIN 913 M4 x 4:2
- Passend:409 [Mate]: 16221600:1 ↔ DIN 913 M4 x 4:1
- Passend:410 [Mate]: Übertragung des Zahnriemens:1 ↔ BS EN ISO 13337 3 x 20:1
- Passend:411 [Mate]: Übertragung des Zahnriemens:1 ↔ DIN 913 M4 x 4:3
- Passend:413 [Mate]: CoverBase_r1:1 ↔ DIN 711 511 20 - 100 x 135 x 25:1
- Passend:414 [Mate]: CoverBase_r1:1 ↔ DIN 711 511 20 - 100 x 135 x 25:1
- Passend:415 [Mate]: CoverBase_r1:1 ↔ DIN 625 SKF SKF 61818:3
- Passend:416 [Mate]: CoverBase_r1:1 ↔ DIN 625 SKF SKF 61818:3
- Fluchtend:59 [Flush]: DIN 912 - ersetzt durch DIN EN ISO 4762 M4 x 50:13 ↔ DIN 912 - ersetzt durch DIN EN ISO 4762 M4 x 50:17
- Passend:418 [Mate]: CoverBase_r1:1 ↔ encoderR1_mini:1
- Passend:419 [Mate]: CoverBase_r1:1
- Passend:420 [Mate]: CoverBase_r1:1 ↔ encoderR1_mini:1
- Passend:421 [Mate]: CoverBase_r1:1 ↔ encoderR1_mini:1
- Passend:422 [Mate]: Übertragung des Zahnriemens:1 ↔ encoder_neu:1
- Passend:423 [Mate]: Shoulder_basis_N24:1 ↔ encoder_neu:1
- Passend:424 [Mate]: Shoulder_basis_N24:1 ↔ encoder_neu:1
- Passend:425 [Mate]: Shoulder_basis_N24:1 ↔ DIN 912 - ersetzt durch DIN EN ISO 4762 M4 x 60:1
- Passend:426 [Mate]: Shoulder_basis_N24:1 ↔ DIN 912 - ersetzt durch DIN EN ISO 4762 M4 x 60:1
- Passend:427 [Mate]: CoverBase_r1:1 ↔ DIN 912 - ersetzt durch DIN EN ISO 4762 M4 x 40:2
- [Mate]: DIN 912 - ersetzt durch DIN EN ISO 4762 M4 x 40:2 ↔ DIN 9021 4,3:11
- [Mate]: DIN 912 - ersetzt durch DIN EN ISO 4762 M4 x 40:2 ↔ DIN 9021 4,3:11
- Passend:430 [Mate]: CoverBase_r1:1 ↔ DIN 9021 4,3:11
- Passend:431 [Mate]: DIN 912 - ersetzt durch DIN EN ISO 4762 M4 x 40:2 ↔ Distanzhuelse_M4x20mm:13
- [Mate]: DIN 912 - ersetzt durch DIN EN ISO 4762 M4 x 40:3 ↔ DIN 9021 4,3:12
- [Mate]: DIN 912 - ersetzt durch DIN EN ISO 4762 M4 x 40:3 ↔ DIN 9021 4,3:12
- [Mate]: DIN 912 - ersetzt durch DIN EN ISO 4762 M4 x 40:3 ↔ Distanzhuelse_M4x20mm:14
- Passend:435 [Mate]: DIN 912 - ersetzt durch DIN EN ISO 4762 M4 x 60:20 ↔ Distanzhuelse_M4x20mm:14
- Fluchtend:60 [Flush]: Distanzhuelse_M4x20mm:13 ↔ Distanzhuelse_M4x20mm:14
- Fluchtend:61 [Flush]: DIN 9021 4,3:11 ↔ DIN 9021 4,3:12
- Fluchtend:62 [Flush]: DIN 912 - ersetzt durch DIN EN ISO 4762 M4 x 60:1 ↔ DIN 912 - ersetzt durch DIN EN ISO 4762 M4 x 60:20
- [Mate]: DIN 912 - ersetzt durch DIN EN ISO 4762 M4 x 40:4 ↔ DIN 9021 4,3:13
- [Mate]: DIN 912 - ersetzt durch DIN EN ISO 4762 M4 x 40:4 ↔ DIN 9021 4,3:13
- [Mate]: DIN 912 - ersetzt durch DIN EN ISO 4762 M4 x 40:4 ↔ Distanzhuelse_M4x20mm:15
- [Mate]: DIN 912 - ersetzt durch DIN EN ISO 4762 M4 x 60:21 ↔ Distanzhuelse_M4x20mm:15
- [Mate]: DIN 912 - ersetzt durch DIN EN ISO 4762 M4 x 40:5 ↔ DIN 9021 4,3:14
- [Mate]: DIN 912 - ersetzt durch DIN EN ISO 4762 M4 x 40:5 ↔ DIN 9021 4,3:14
- [Mate]: DIN 912 - ersetzt durch DIN EN ISO 4762 M4 x 40:5 ↔ Distanzhuelse_M4x20mm:16
- [Mate]: DIN 912 - ersetzt durch DIN EN ISO 4762 M4 x 60:22 ↔ Distanzhuelse_M4x20mm:16
- [Mate]: DIN 912 - ersetzt durch DIN EN ISO 4762 M4 x 40:6 ↔ DIN 9021 4,3:15
- [Mate]: DIN 912 - ersetzt durch DIN EN ISO 4762 M4 x 40:6 ↔ DIN 9021 4,3:15
- [Mate]: DIN 912 - ersetzt durch DIN EN ISO 4762 M4 x 40:6 ↔ Distanzhuelse_M4x20mm:17
- [Mate]: DIN 912 - ersetzt durch DIN EN ISO 4762 M4 x 60:23 ↔ Distanzhuelse_M4x20mm:17
- Passend:448 [Mate]: Shoulder_basis_N24:1 ↔ DIN 912 - ersetzt durch DIN EN ISO 4762 M4 x 60:20
- Passend:449 [Mate]: Shoulder_basis_N24:1 ↔ DIN 912 - ersetzt durch DIN EN ISO 4762 M4 x 60:23
- Passend:450 [Mate]: Shoulder_basis_N24:1 ↔ DIN 912 - ersetzt durch DIN EN ISO 4762 M4 x 60:22
- Passend:451 [Mate]: Shoulder_basis_N24:1 ↔ DIN 912 - ersetzt durch DIN EN ISO 4762 M4 x 60:21
- [Mate]: DIN 912 - ersetzt durch DIN EN ISO 4762 M4 x 40:7 ↔ DIN 9021 4,3:16
- [Mate]: DIN 912 - ersetzt durch DIN EN ISO 4762 M4 x 40:7 ↔ DIN 9021 4,3:16
- [Mate]: DIN 912 - ersetzt durch DIN EN ISO 4762 M4 x 40:7 ↔ Distanzhuelse_M4x20mm:18
- [Mate]: DIN 912 - ersetzt durch DIN EN ISO 4762 M4 x 60:24 ↔ Distanzhuelse_M4x20mm:18
- Passend:456 [Mate]: Shoulder_basis_N24:1 ↔ DIN 912 - ersetzt durch DIN EN ISO 4762 M4 x 60:24
- Fluchtend:63 [Flush]: DIN 912 - ersetzt durch DIN EN ISO 4762 M4 x 60:22 ↔ DIN 912 - ersetzt durch DIN EN ISO 4762 M4 x 60:24
- Fluchtend:64 [Flush]: DIN 912 - ersetzt durch DIN EN ISO 4762 M4 x 60:21 ↔ DIN 912 - ersetzt durch DIN EN ISO 4762 M4 x 60:24
- Fluchtend:65 [Flush]: DIN 912 - ersetzt durch DIN EN ISO 4762 M4 x 60:21 ↔ DIN 912 - ersetzt durch DIN EN ISO 4762 M4 x 60:23
- Fluchtend:66 [Flush]: DIN 912 - ersetzt durch DIN EN ISO 4762 M4 x 60:1 ↔ DIN 912 - ersetzt durch DIN EN ISO 4762 M4 x 60:23
- Fluchtend:67 [Flush]: Distanzhuelse_M4x20mm:13 ↔ Distanzhuelse_M4x20mm:17
- Fluchtend:68 [Flush]: Distanzhuelse_M4x20mm:13 ↔ Distanzhuelse_M4x20mm:18
- Fluchtend:69 [Flush]: Distanzhuelse_M4x20mm:16 ↔ Distanzhuelse_M4x20mm:18
- Fluchtend:70 [Flush]: Distanzhuelse_M4x20mm:15 ↔ Distanzhuelse_M4x20mm:18
- Fluchtend:71 [Flush]: DIN 9021 4,3:13 ↔ DIN 9021 4,3:16
- Fluchtend:72 [Flush]: DIN 9021 4,3:14 ↔ DIN 9021 4,3:16
- Fluchtend:73 [Flush]: DIN 9021 4,3:11 ↔ DIN 9021 4,3:14
- Fluchtend:74 [Flush]: DIN 9021 4,3:11 ↔ DIN 9021 4,3:12
- Fluchtend:75 [Flush]: DIN 9021 4,3:11 ↔ DIN 9021 4,3:15
- Passend:457 [Mate]: CoverBase_r1:1 ↔ DIN 912 - ersetzt durch DIN EN ISO 4762 M4 x 30:4
- Passend:458 [Mate]: CoverBase_r1:1 ↔ DIN 912 - ersetzt durch DIN EN ISO 4762 M4 x 30:3
- Passend:459 [Mate]: Nema24_100:1 ↔ DIN 912 - ersetzt durch DIN EN ISO 4762 M4 x 30:4
- Passend:460 [Mate]: Nema24_100:1 ↔ DIN 912 - ersetzt durch DIN EN ISO 4762 M4 x 30:3
- Passend:461 [Mate]: DIN 912 - ersetzt durch DIN EN ISO 4762 M4 x 30:3 ↔ DIN 934 - ersetzt durch DIN EN 24032/28673/28674 M4:19
- Passend:462 [Mate]: DIN 912 - ersetzt durch DIN EN ISO 4762 M4 x 30:4 ↔ DIN 934 - ersetzt durch DIN EN 24032/28673/28674 M4:20
- Fluchtend:76 [Flush]: DIN 934 - ersetzt durch DIN EN 24032/28673/28674 M4:19 ↔ DIN 934 - ersetzt durch DIN EN 24032/28673/28674 M4:20
- Fluchtend:77 [Flush]: DIN 934 - ersetzt durch DIN EN 24032/28673/28674 M4:19 ↔ DIN 934 - ersetzt durch DIN EN 24032/28673/28674 M4:20
- Passend:463 [Mate]: CoverBase_r1:1 ↔ DIN 125-1 A A 4,3:18
- Passend:464 [Mate]: Nema24_100:1 ↔ Nema23_24Mount:1
- Passend:465 [Mate]: Nema24_100:1 ↔ Nema23_24Mount:1
- Passend:466 [Mate]: Nema24_100:1 ↔ Nema23_24Mount:1
- Passend:467 [Mate]: Nema24_100:1 ↔ Nema23_24Mount:2
- Passend:468 [Mate]: DIN 912 - ersetzt durch DIN EN ISO 4762 M4 x 20:5 ↔ Nema23_24Mount:2
- Passend:469 [Mate]: Nema24_100:1 ↔ DIN 912 - ersetzt durch DIN EN ISO 4762 M4 x 20:5
- Passend:470 [Mate]: DIN 912 - ersetzt durch DIN EN ISO 4762 M4 x 20:4 ↔ Nema23_24Mount:2
- Passend:471 [Mate]: Nema24_100:1 ↔ DIN 912 - ersetzt durch DIN EN ISO 4762 M4 x 20:4
- Passend:472 [Mate]: CoverBase_r1:1 ↔ DIN 912 - ersetzt durch DIN EN ISO 4762 M4 x 30:5
## Named parameters: d574_d570 = 0 mm, d575_d573 = 0 mm, d576_d571 = 0 mm, d581_d574_d570 = 0 mm, d582_d575_d573 = 0 mm, d583_d576_d571 = 0 mm, d584_d577 = 0 mm, d585_d574_d570 = 0 mm, d586_d575_d573 = 0 mm, d587_d576_d571 = 0 mm, d588_d577 = 0 mm, d589_d574_d570 = 0 mm, d590_d575_d573 = 0 mm, d591_d576_d571 = 0 mm, d592_d577 = 0 mm, d597_d574_d570 = 0 mm, d598_d575_d573 = 0 mm, d599_d576_d571 = 0 mm, d600_d577 = 0 mm
